# Autodesk Inventor assembly: 하단부 뚜껑
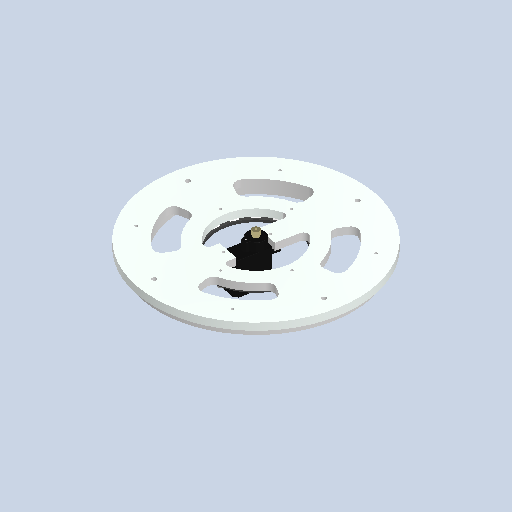
[picture p0: Inventor's stored thumbnail of the model, 512x512]
Saved by Autodesk Inventor 2023 (Build 270158000, 158)
## iProperties
Created: 2022-06-06
Part Number: 하단부 뚜껑
Document SubType Name: Assembly
Designer: fly01
Author: fly01
## Documents named in this file (6)
- C:\Users\fly01\Desktop\2022카이스트 입학준비\스마트홈\제작부품'\하단부 뚜껑.iam
- C:\Users\fly01\Desktop\2022카이스트 입학준비\스마트홈\범용 부품\Neopixel circle.ipt
- C:\Users\fly01\Desktop\2022카이스트 입학준비\스마트홈\범용 부품\부속부품 2. 180도 서보모터.ipt
- C:\Users\fly01\Desktop\2022카이스트 입학준비\스마트홈\제작부품'\아크릴 빛번짐 고정용.ipt
- C:\Users\fly01\Desktop\2022카이스트 입학준비\스마트홈\제작부품'\아크릴 빛번짐.ipt
- C:\Users\fly01\Desktop\2022카이스트 입학준비\스마트홈\범용 부품\십자 둥근머리 볼트 6mm.ipt
## Components (10 placed, 5 different names)
1. Neopixel circle:1 — 회전:1, 삽입:6, 삽입:7, 삽입:8, 삽입:9
2. 부속부품 2. 180도 서보모터:1 — 삽입:10, 삽입:11, 삽입:13, 삽입:14
3. 아크릴 빛번짐 고정용:1 — 삽입:4, 삽입:5
4. 아크릴 빛번짐:1 — 회전:1, 삽입:4, 삽입:5, 삽입:10, 삽입:11
5. 십자 둥근머리 볼트 6mm:1 — 삽입:6
6. 십자 둥근머리 볼트 6mm:2 — 삽입:7
7. 십자 둥근머리 볼트 6mm:3 — 삽입:8
8. 십자 둥근머리 볼트 6mm:4 — 삽입:9
9. 십자 둥근머리 볼트 6mm:5 — 삽입:13
10. 십자 둥근머리 볼트 6mm:6 — 삽입:14
## Relationships (11: Insert 10, RevoluteJoint 1)
- 회전:1 [RevoluteJoint] (-1.7 mm): Neopixel circle:1 ↔ 아크릴 빛번짐:1
- 삽입:4 [Insert]: 아크릴 빛번짐 고정용:1 ↔ 아크릴 빛번짐:1
- 삽입:5 [Insert]: 아크릴 빛번짐 고정용:1 ↔ 아크릴 빛번짐:1
- 삽입:6 [Insert]: Neopixel circle:1 ↔ 십자 둥근머리 볼트 6mm:1
- 삽입:7 [Insert]: Neopixel circle:1 ↔ 십자 둥근머리 볼트 6mm:2
- 삽입:8 [Insert]: Neopixel circle:1 ↔ 십자 둥근머리 볼트 6mm:3
- 삽입:9 [Insert]: Neopixel circle:1 ↔ 십자 둥근머리 볼트 6mm:4
- 삽입:10 [Insert]: 부속부품 2. 180도 서보모터:1 ↔ 아크릴 빛번짐:1
- 삽입:11 [Insert]: 부속부품 2. 180도 서보모터:1 ↔ 아크릴 빛번짐:1
- 삽입:13 [Insert]: 부속부품 2. 180도 서보모터:1 ↔ 십자 둥근머리 볼트 6mm:5
- 삽입:14 [Insert]: 부속부품 2. 180도 서보모터:1 ↔ 십자 둥근머리 볼트 6mm:6
